# Autodesk Inventor assembly: gearset_fin
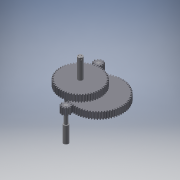
[picture p0: Inventor's stored thumbnail of the model, 180x180]
Saved by Autodesk Inventor 2016 SP1 (Build 200210100, 210)
## iProperties
Created: 2017-01-25
Part Number: gearset_fin
Material: 一般
Document SubType Name: Assembly
Designer: p_admin
Author: p_admin
## Documents named in this file (4)
- Z:\風力発電機\gearset_fin.iam
- Z:\風力発電機\gear_60.iam
- Z:\風力発電機\gear_72.iam
- Z:\風力発電機\gear_shaft.ipt
## Components (3 placed, 3 different names)
1. gear_60:1 [sub-assembly] — 回転:1
2. gear_72:1 [sub-assembly] — 回転:1, 回転:2
3. gear_shaft:1 — 回転:2
## Relationships (2: RevoluteJoint 2)
- 回転:1 [RevoluteJoint]: gear_60:1 ↔ gear_72:1
- 回転:2 [RevoluteJoint]: gear_72:1 ↔ gear_shaft:1
